# Autodesk Inventor assembly: BevelSystem
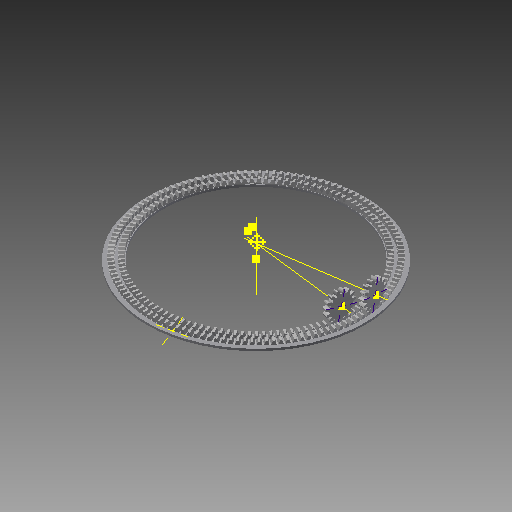
[picture p0: Inventor's stored thumbnail of the model, 512x512]
Saved by Autodesk Inventor 2017 (Build 210142000, 142)
## iProperties
Created: 2017-01-10
Part Number: BevelSystem
Document SubType Name: Assembly
Designer: David Kopala
Author: David Kopala
## Documents named in this file (4)
- Z:\Documents\Drone\Drone\3D Models\Project\Chasis_03\BevelSystem.iam
- Z:\Documents\Drone\Drone\3D Models\Project\Chasis_03\Bevel_BasePlate.ipt
- Z:\Documents\Drone\Drone\3D Models\Project\Chasis_03\Bevel_Outer_Reference.iam
- Z:\Documents\Drone\Drone\3D Models\Project\Chasis_03\Bevel_Inner_Reference.iam
## Components (4 placed, 3 different names)
1. Bevel_BasePlate:1 — Mate:2, Mate:3, Insert:1, Insert:2, Mate:4
2. Bevel_Outer_Reference:1 [sub-assembly] — Mate:2, Insert:2
3. Bevel_Inner_Reference:1 [sub-assembly] — Mate:3, Insert:1, Insert:3
4. Bevel_Inner_Reference:2 [sub-assembly] — Mate:4, Insert:3
## Relationships (6: Mate 3, Insert 3)
- Mate:2: Bevel_BasePlate:1 ↔ Bevel_Outer_Reference:1
- Mate:3: Bevel_BasePlate:1 ↔ Bevel_Inner_Reference:1
- Insert:1: Bevel_BasePlate:1 ↔ Bevel_Inner_Reference:1
- Insert:2: Bevel_BasePlate:1 ↔ Bevel_Outer_Reference:1
- Mate:4: Bevel_BasePlate:1 ↔ Bevel_Inner_Reference:2
- Insert:3: Bevel_Inner_Reference:1 ↔ Bevel_Inner_Reference:2
